# Autodesk Inventor assembly: NewAssembly
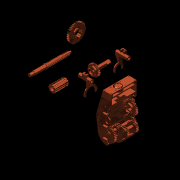
[picture p0: Inventor's stored thumbnail of the model, 180x180]
Saved by Autodesk Inventor 2022 (Build 260153000, 153)
## iProperties
Created: 2021-07-18
Part Number: NewAssembly
Document SubType Name: Assembly
Designer: jdski
Author: jdski
## Documents named in this file (15)
- C:\Users\jdski\Documents\Inventor\Eng312Project\NewStart\NewAssembly.iam
- C:\Users\jdski\Documents\Inventor\Eng312Project\NewStart\CaseLid.ipt
- C:\Users\jdski\Documents\Inventor\Eng312Project\NewStart\ShftHldrLH.ipt
- C:\Users\jdski\Documents\Inventor\Eng312Project\NewStart\ShftHldrRH.ipt
- C:\Users\jdski\Documents\Inventor\Eng312Project\NewStart\CaseFinal.ipt
- C:\Users\jdski\Documents\Inventor\Eng312Project\NewStart\GearPawl.ipt
- C:\Users\jdski\Documents\Inventor\Eng312Project\NewStart\InputShaftGear0.ipt
- C:\Users\jdski\Documents\Inventor\Eng312Project\NewStart\OutputGear5.ipt
- C:\Users\jdski\Documents\Inventor\Eng312Project\NewStart\OutputShaft.ipt
- C:\Users\jdski\Documents\Inventor\Eng312Project\NewStart\ShiftBall.ipt
- C:\Users\jdski\Documents\Inventor\Eng312Project\NewStart\SplinedSleeve.ipt
- C:\Users\jdski\Documents\Inventor\Eng312Project\NewStart\SleevePawl.ipt
- C:\Users\jdski\Documents\Inventor\Eng312Project\NewStart\ShiftGear3.ipt
- C:\Users\jdski\Documents\Inventor\Eng312Project\NewStart\IdlerShaft.ipt
- C:\Users\jdski\Documents\Inventor\Eng312Project\NewStart\LayShaft.ipt
## Components (14 placed, 14 different names)
1. CaseLid:1
2. ShftHldrLH:1
3. ShftHldrRH:1
4. CaseFinal:1 — Ball:1, Rotational:1, Rotational:2, Rotational:3
5. GearPawl:1
6. InputShaftGear0:1
7. OutputGear5:1 — Rotational:3
8. OutputShaft:1
9. ShiftBall:1 — Ball:1
10. SplinedSleeve:1
11. SleevePawl:1
12. ShiftGear3:1
13. IdlerShaft:1 — Rotational:2
14. LayShaft:1 — Rotational:1
## Relationships (4: RevoluteJoint 3, BallJoint 1)
- Ball:1: CaseFinal:1 ↔ ShiftBall:1
- Rotational:1 [RevoluteJoint]: CaseFinal:1 ↔ LayShaft:1
- Rotational:2 [RevoluteJoint]: CaseFinal:1 ↔ IdlerShaft:1
- Rotational:3 [RevoluteJoint]: CaseFinal:1 ↔ OutputGear5:1
